# Autodesk Inventor assembly: platform_0606_fig2_ratio10
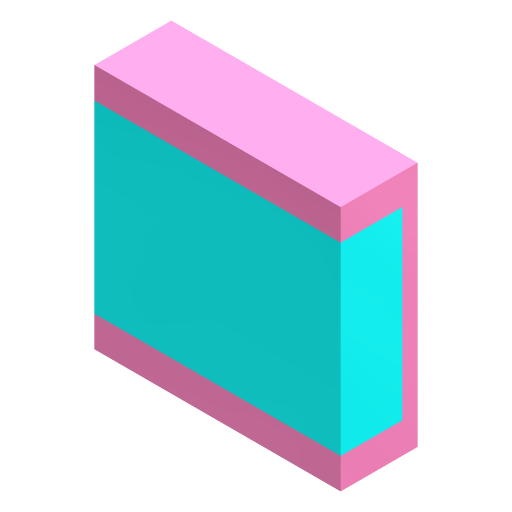
[picture p0: Inventor's stored thumbnail of the model, 512x512]
Saved by Autodesk Inventor 2024 (Build 280153000, 153)
## iProperties
Created: 2024-06-06
Part Number: platform_0606_fig2_ratio10
Document SubType Name: Assembly
Designer: admin
Author: admin
## Documents named in this file (3)
- C:\Users\admin\OneDrive\文件\碩士研究\prototype\plane_unit_0606\platform_0606_fig1_ratio10_with_support.iam
- C:\Users\admin\OneDrive\文件\碩士研究\prototype\plane_unit_0606\bridge_rect_final_10.ipt
- C:\Users\admin\OneDrive\文件\碩士研究\prototype\plane_unit_0606\support_ratio10.ipt
## Components (2 placed, 2 different names)
1. bridge_rect_final_10:1 — 齊平:3, 貼合:2, 貼合:3
2. support_ratio10:1 — 齊平:3, 貼合:2, 貼合:3
## Relationships (3: Mate 2, Flush 1)
- 齊平:3 [Flush]: bridge_rect_final_10:1 ↔ support_ratio10:1
- 貼合:2 [Mate]: bridge_rect_final_10:1 ↔ support_ratio10:1
- 貼合:3 [Mate]: bridge_rect_final_10:1 ↔ support_ratio10:1
